(part 1 of 2)
# Autodesk Inventor assembly: Raspberry_Pi4 v19
Saved by Autodesk Inventor 2021.3 (Build 253353000, 353)
## iProperties
Created: 2023-06-15
Part Number: Raspberry_Pi4 v19
Document SubType Name: Assembly
Designer: AdminForWorker
Title: Raspberry_Pi4 v19 v1
Author: AdminForWorker
## Documents named in this file (370)
- z:\worker\convert-fusion-r02-cosv3\tmp\job-1\86\output\files\932a8257-b544-4e70-8857-ce00fc62fffb\fd29544b-6eeb-4b26-ae93-db3abaadae4f.iam
- z:\worker\convert-fusion-r02-cosv3\tmp\job-1\86\output\files\932a8257-b544-4e70-8857-ce00fc62fffb\Raspberry Pi 3157.ipt
- z:\worker\convert-fusion-r02-cosv3\tmp\job-1\86\output\files\932a8257-b544-4e70-8857-ce00fc62fffb\Raspberry Pi 3236.ipt
- z:\worker\convert-fusion-r02-cosv3\tmp\job-1\86\output\files\932a8257-b544-4e70-8857-ce00fc62fffb\Raspberry Pi 3237.ipt
- z:\worker\convert-fusion-r02-cosv3\tmp\job-1\86\output\files\932a8257-b544-4e70-8857-ce00fc62fffb\Raspberry Pi 3238.ipt
- z:\worker\convert-fusion-r02-cosv3\tmp\job-1\86\output\files\932a8257-b544-4e70-8857-ce00fc62fffb\Raspberry Pi 3239.ipt
- z:\worker\convert-fusion-r02-cosv3\tmp\job-1\86\output\files\932a8257-b544-4e70-8857-ce00fc62fffb\Raspberry Pi 3240.ipt
- z:\worker\convert-fusion-r02-cosv3\tmp\job-1\86\output\files\932a8257-b544-4e70-8857-ce00fc62fffb\Raspberry Pi 3241.ipt
- z:\worker\convert-fusion-r02-cosv3\tmp\job-1\86\output\files\932a8257-b544-4e70-8857-ce00fc62fffb\Raspberry Pi 3242.ipt
- z:\worker\convert-fusion-r02-cosv3\tmp\job-1\86\output\files\932a8257-b544-4e70-8857-ce00fc62fffb\Raspberry Pi 3243.ipt
- z:\worker\convert-fusion-r02-cosv3\tmp\job-1\86\output\files\932a8257-b544-4e70-8857-ce00fc62fffb\Raspberry Pi 3244.ipt
- z:\worker\convert-fusion-r02-cosv3\tmp\job-1\86\output\files\932a8257-b544-4e70-8857-ce00fc62fffb\Raspberry Pi 3245.ipt
- z:\worker\convert-fusion-r02-cosv3\tmp\job-1\86\output\files\932a8257-b544-4e70-8857-ce00fc62fffb\Raspberry Pi 3246.ipt
- z:\worker\convert-fusion-r02-cosv3\tmp\job-1\86\output\files\932a8257-b544-4e70-8857-ce00fc62fffb\Raspberry Pi 3247.ipt
- z:\worker\convert-fusion-r02-cosv3\tmp\job-1\86\output\files\932a8257-b544-4e70-8857-ce00fc62fffb\Raspberry Pi 3248.ipt
- z:\worker\convert-fusion-r02-cosv3\tmp\job-1\86\output\files\932a8257-b544-4e70-8857-ce00fc62fffb\Raspberry Pi 3249.ipt
- z:\worker\convert-fusion-r02-cosv3\tmp\job-1\86\output\files\932a8257-b544-4e70-8857-ce00fc62fffb\Raspberry Pi 3250.ipt
- z:\worker\convert-fusion-r02-cosv3\tmp\job-1\86\output\files\932a8257-b544-4e70-8857-ce00fc62fffb\Raspberry Pi 3251.ipt
- z:\worker\convert-fusion-r02-cosv3\tmp\job-1\86\output\files\932a8257-b544-4e70-8857-ce00fc62fffb\Raspberry Pi 3252.ipt
- z:\worker\convert-fusion-r02-cosv3\tmp\job-1\86\output\files\932a8257-b544-4e70-8857-ce00fc62fffb\Raspberry Pi 3253.ipt
- z:\worker\convert-fusion-r02-cosv3\tmp\job-1\86\output\files\932a8257-b544-4e70-8857-ce00fc62fffb\Raspberry Pi 3254.ipt
- z:\worker\convert-fusion-r02-cosv3\tmp\job-1\86\output\files\932a8257-b544-4e70-8857-ce00fc62fffb\Raspberry Pi 3255.ipt
- z:\worker\convert-fusion-r02-cosv3\tmp\job-1\86\output\files\932a8257-b544-4e70-8857-ce00fc62fffb\Raspberry Pi 3256.ipt
- z:\worker\convert-fusion-r02-cosv3\tmp\job-1\86\output\files\932a8257-b544-4e70-8857-ce00fc62fffb\Raspberry Pi 3257.ipt
- z:\worker\convert-fusion-r02-cosv3\tmp\job-1\86\output\files\932a8257-b544-4e70-8857-ce00fc62fffb\Raspberry Pi 3258.ipt
- z:\worker\convert-fusion-r02-cosv3\tmp\job-1\86\output\files\932a8257-b544-4e70-8857-ce00fc62fffb\Raspberry Pi 3259.ipt
- z:\worker\convert-fusion-r02-cosv3\tmp\job-1\86\output\files\932a8257-b544-4e70-8857-ce00fc62fffb\Raspberry Pi 3260.ipt
- z:\worker\convert-fusion-r02-cosv3\tmp\job-1\86\output\files\932a8257-b544-4e70-8857-ce00fc62fffb\Raspberry Pi 3261.ipt
- z:\worker\convert-fusion-r02-cosv3\tmp\job-1\86\output\files\932a8257-b544-4e70-8857-ce00fc62fffb\Raspberry Pi 3262.ipt
- z:\worker\convert-fusion-r02-cosv3\tmp\job-1\86\output\files\932a8257-b544-4e70-8857-ce00fc62fffb\Raspberry Pi 3263.ipt
- z:\worker\convert-fusion-r02-cosv3\tmp\job-1\86\output\files\932a8257-b544-4e70-8857-ce00fc62fffb\Raspberry Pi 3264.ipt
- z:\worker\convert-fusion-r02-cosv3\tmp\job-1\86\output\files\932a8257-b544-4e70-8857-ce00fc62fffb\Raspberry Pi 3265.ipt
- z:\worker\convert-fusion-r02-cosv3\tmp\job-1\86\output\files\932a8257-b544-4e70-8857-ce00fc62fffb\Raspberry Pi 3266.ipt
- z:\worker\convert-fusion-r02-cosv3\tmp\job-1\86\output\files\932a8257-b544-4e70-8857-ce00fc62fffb\Raspberry Pi 3267.ipt
- z:\worker\convert-fusion-r02-cosv3\tmp\job-1\86\output\files\932a8257-b544-4e70-8857-ce00fc62fffb\Raspberry Pi 3268.ipt
- z:\worker\convert-fusion-r02-cosv3\tmp\job-1\86\output\files\932a8257-b544-4e70-8857-ce00fc62fffb\Raspberry Pi 3269.ipt
- z:\worker\convert-fusion-r02-cosv3\tmp\job-1\86\output\files\932a8257-b544-4e70-8857-ce00fc62fffb\Raspberry Pi 3270.ipt
- z:\worker\convert-fusion-r02-cosv3\tmp\job-1\86\output\files\932a8257-b544-4e70-8857-ce00fc62fffb\Raspberry Pi 3271.ipt
- z:\worker\convert-fusion-r02-cosv3\tmp\job-1\86\output\files\932a8257-b544-4e70-8857-ce00fc62fffb\Raspberry Pi 3272.ipt
- z:\worker\convert-fusion-r02-cosv3\tmp\job-1\86\output\files\932a8257-b544-4e70-8857-ce00fc62fffb\Raspberry Pi 3273.ipt
- z:\worker\convert-fusion-r02-cosv3\tmp\job-1\86\output\files\932a8257-b544-4e70-8857-ce00fc62fffb\Raspberry Pi 3274.ipt
- z:\worker\convert-fusion-r02-cosv3\tmp\job-1\86\output\files\932a8257-b544-4e70-8857-ce00fc62fffb\Raspberry Pi 3275.ipt
- z:\worker\convert-fusion-r02-cosv3\tmp\job-1\86\output\files\932a8257-b544-4e70-8857-ce00fc62fffb\RPi3_ModelB v1.iam
- z:\worker\convert-fusion-r02-cosv3\tmp\job-1\86\output\files\932a8257-b544-4e70-8857-ce00fc62fffb\Raspberry Pi 312.ipt
- z:\worker\convert-fusion-r02-cosv3\tmp\job-1\86\output\files\932a8257-b544-4e70-8857-ce00fc62fffb\Raspberry Pi 314.ipt
- z:\worker\convert-fusion-r02-cosv3\tmp\job-1\86\output\files\932a8257-b544-4e70-8857-ce00fc62fffb\Raspberry Pi 3172.ipt
- z:\worker\convert-fusion-r02-cosv3\tmp\job-1\86\output\files\932a8257-b544-4e70-8857-ce00fc62fffb\Raspberry Pi 3173.ipt
- z:\worker\convert-fusion-r02-cosv3\tmp\job-1\86\output\files\932a8257-b544-4e70-8857-ce00fc62fffb\Raspberry Pi 3174.ipt
- z:\worker\convert-fusion-r02-cosv3\tmp\job-1\86\output\files\932a8257-b544-4e70-8857-ce00fc62fffb\Raspberry Pi 3175.ipt
- z:\worker\convert-fusion-r02-cosv3\tmp\job-1\86\output\files\932a8257-b544-4e70-8857-ce00fc62fffb\Raspberry Pi 3176.ipt
- z:\worker\convert-fusion-r02-cosv3\tmp\job-1\86\output\files\932a8257-b544-4e70-8857-ce00fc62fffb\Raspberry Pi 3177.ipt
- z:\worker\convert-fusion-r02-cosv3\tmp\job-1\86\output\files\932a8257-b544-4e70-8857-ce00fc62fffb\Raspberry Pi 3178.ipt
- z:\worker\convert-fusion-r02-cosv3\tmp\job-1\86\output\files\932a8257-b544-4e70-8857-ce00fc62fffb\Raspberry Pi 3179.ipt
- z:\worker\convert-fusion-r02-cosv3\tmp\job-1\86\output\files\932a8257-b544-4e70-8857-ce00fc62fffb\Raspberry Pi 3180.ipt
- z:\worker\convert-fusion-r02-cosv3\tmp\job-1\86\output\files\932a8257-b544-4e70-8857-ce00fc62fffb\Raspberry Pi 3181.ipt
- z:\worker\convert-fusion-r02-cosv3\tmp\job-1\86\output\files\932a8257-b544-4e70-8857-ce00fc62fffb\Raspberry Pi 3182.ipt
- z:\worker\convert-fusion-r02-cosv3\tmp\job-1\86\output\files\932a8257-b544-4e70-8857-ce00fc62fffb\Raspberry Pi 3183.ipt
- z:\worker\convert-fusion-r02-cosv3\tmp\job-1\86\output\files\932a8257-b544-4e70-8857-ce00fc62fffb\Raspberry Pi 3184.ipt
- z:\worker\convert-fusion-r02-cosv3\tmp\job-1\86\output\files\932a8257-b544-4e70-8857-ce00fc62fffb\Raspberry Pi 3185.ipt
- z:\worker\convert-fusion-r02-cosv3\tmp\job-1\86\output\files\932a8257-b544-4e70-8857-ce00fc62fffb\Raspberry Pi 3186.ipt
- z:\worker\convert-fusion-r02-cosv3\tmp\job-1\86\output\files\932a8257-b544-4e70-8857-ce00fc62fffb\Raspberry Pi 3187.ipt
- z:\worker\convert-fusion-r02-cosv3\tmp\job-1\86\output\files\932a8257-b544-4e70-8857-ce00fc62fffb\Raspberry Pi 3188.ipt
- z:\worker\convert-fusion-r02-cosv3\tmp\job-1\86\output\files\932a8257-b544-4e70-8857-ce00fc62fffb\Raspberry Pi 3189.ipt
- z:\worker\convert-fusion-r02-cosv3\tmp\job-1\86\output\files\932a8257-b544-4e70-8857-ce00fc62fffb\Raspberry Pi 3190.ipt
- z:\worker\convert-fusion-r02-cosv3\tmp\job-1\86\output\files\932a8257-b544-4e70-8857-ce00fc62fffb\Raspberry Pi 3191.ipt
- z:\worker\convert-fusion-r02-cosv3\tmp\job-1\86\output\files\932a8257-b544-4e70-8857-ce00fc62fffb\Raspberry Pi 3192.ipt
- z:\worker\convert-fusion-r02-cosv3\tmp\job-1\86\output\files\932a8257-b544-4e70-8857-ce00fc62fffb\Raspberry Pi 3193.ipt
- z:\worker\convert-fusion-r02-cosv3\tmp\job-1\86\output\files\932a8257-b544-4e70-8857-ce00fc62fffb\Raspberry Pi 3194.ipt
- z:\worker\convert-fusion-r02-cosv3\tmp\job-1\86\output\files\932a8257-b544-4e70-8857-ce00fc62fffb\Raspberry Pi 3195.ipt
- z:\worker\convert-fusion-r02-cosv3\tmp\job-1\86\output\files\932a8257-b544-4e70-8857-ce00fc62fffb\Raspberry Pi 3196.ipt
- z:\worker\convert-fusion-r02-cosv3\tmp\job-1\86\output\files\932a8257-b544-4e70-8857-ce00fc62fffb\Raspberry Pi 3197.ipt
- z:\worker\convert-fusion-r02-cosv3\tmp\job-1\86\output\files\932a8257-b544-4e70-8857-ce00fc62fffb\Raspberry Pi 3198.ipt
- z:\worker\convert-fusion-r02-cosv3\tmp\job-1\86\output\files\932a8257-b544-4e70-8857-ce00fc62fffb\Raspberry Pi 3199.ipt
- z:\worker\convert-fusion-r02-cosv3\tmp\job-1\86\output\files\932a8257-b544-4e70-8857-ce00fc62fffb\Raspberry Pi 3200.ipt
- z:\worker\convert-fusion-r02-cosv3\tmp\job-1\86\output\files\932a8257-b544-4e70-8857-ce00fc62fffb\Raspberry Pi 3201.ipt
- z:\worker\convert-fusion-r02-cosv3\tmp\job-1\86\output\files\932a8257-b544-4e70-8857-ce00fc62fffb\Raspberry Pi 3202.ipt
- z:\worker\convert-fusion-r02-cosv3\tmp\job-1\86\output\files\932a8257-b544-4e70-8857-ce00fc62fffb\Raspberry Pi 3203.ipt
- z:\worker\convert-fusion-r02-cosv3\tmp\job-1\86\output\files\932a8257-b544-4e70-8857-ce00fc62fffb\Raspberry Pi 3204.ipt
- z:\worker\convert-fusion-r02-cosv3\tmp\job-1\86\output\files\932a8257-b544-4e70-8857-ce00fc62fffb\Raspberry Pi 3205.ipt
- z:\worker\convert-fusion-r02-cosv3\tmp\job-1\86\output\files\932a8257-b544-4e70-8857-ce00fc62fffb\Raspberry Pi 3206.ipt
- z:\worker\convert-fusion-r02-cosv3\tmp\job-1\86\output\files\932a8257-b544-4e70-8857-ce00fc62fffb\Raspberry Pi 3207.ipt
- z:\worker\convert-fusion-r02-cosv3\tmp\job-1\86\output\files\932a8257-b544-4e70-8857-ce00fc62fffb\Raspberry Pi 3208.ipt
- z:\worker\convert-fusion-r02-cosv3\tmp\job-1\86\output\files\932a8257-b544-4e70-8857-ce00fc62fffb\Raspberry Pi 3209.ipt
- z:\worker\convert-fusion-r02-cosv3\tmp\job-1\86\output\files\932a8257-b544-4e70-8857-ce00fc62fffb\Raspberry Pi 3210.ipt
- z:\worker\convert-fusion-r02-cosv3\tmp\job-1\86\output\files\932a8257-b544-4e70-8857-ce00fc62fffb\Raspberry Pi 3211.ipt
- z:\worker\convert-fusion-r02-cosv3\tmp\job-1\86\output\files\932a8257-b544-4e70-8857-ce00fc62fffb\Raspberry Pi 3212.ipt
- z:\worker\convert-fusion-r02-cosv3\tmp\job-1\86\output\files\932a8257-b544-4e70-8857-ce00fc62fffb\Raspberry Pi 3213.ipt
- z:\worker\convert-fusion-r02-cosv3\tmp\job-1\86\output\files\932a8257-b544-4e70-8857-ce00fc62fffb\Raspberry Pi 3214.ipt
- z:\worker\convert-fusion-r02-cosv3\tmp\job-1\86\output\files\932a8257-b544-4e70-8857-ce00fc62fffb\Raspberry Pi 3215.ipt
- z:\worker\convert-fusion-r02-cosv3\tmp\job-1\86\output\files\932a8257-b544-4e70-8857-ce00fc62fffb\Raspberry Pi 3216.ipt
- z:\worker\convert-fusion-r02-cosv3\tmp\job-1\86\output\files\932a8257-b544-4e70-8857-ce00fc62fffb\Raspberry Pi 3217.ipt
- z:\worker\convert-fusion-r02-cosv3\tmp\job-1\86\output\files\932a8257-b544-4e70-8857-ce00fc62fffb\Raspberry Pi 3218.ipt
- z:\worker\convert-fusion-r02-cosv3\tmp\job-1\86\output\files\932a8257-b544-4e70-8857-ce00fc62fffb\Raspberry Pi 3219.ipt
- z:\worker\convert-fusion-r02-cosv3\tmp\job-1\86\output\files\932a8257-b544-4e70-8857-ce00fc62fffb\Raspberry Pi 3220.ipt
- z:\worker\convert-fusion-r02-cosv3\tmp\job-1\86\output\files\932a8257-b544-4e70-8857-ce00fc62fffb\Raspberry Pi 3221.ipt
- z:\worker\convert-fusion-r02-cosv3\tmp\job-1\86\output\files\932a8257-b544-4e70-8857-ce00fc62fffb\Raspberry Pi 3222.ipt
- z:\worker\convert-fusion-r02-cosv3\tmp\job-1\86\output\files\932a8257-b544-4e70-8857-ce00fc62fffb\Raspberry Pi 3223.ipt
- z:\worker\convert-fusion-r02-cosv3\tmp\job-1\86\output\files\932a8257-b544-4e70-8857-ce00fc62fffb\Raspberry Pi 3224.ipt
- z:\worker\convert-fusion-r02-cosv3\tmp\job-1\86\output\files\932a8257-b544-4e70-8857-ce00fc62fffb\Raspberry Pi 3225.ipt
- z:\worker\convert-fusion-r02-cosv3\tmp\job-1\86\output\files\932a8257-b544-4e70-8857-ce00fc62fffb\Raspberry Pi 3226.ipt
- z:\worker\convert-fusion-r02-cosv3\tmp\job-1\86\output\files\932a8257-b544-4e70-8857-ce00fc62fffb\Raspberry Pi 3227.ipt
- z:\worker\convert-fusion-r02-cosv3\tmp\job-1\86\output\files\932a8257-b544-4e70-8857-ce00fc62fffb\Raspberry Pi 3228.ipt
- z:\worker\convert-fusion-r02-cosv3\tmp\job-1\86\output\files\932a8257-b544-4e70-8857-ce00fc62fffb\Raspberry Pi 3229.ipt
- z:\worker\convert-fusion-r02-cosv3\tmp\job-1\86\output\files\932a8257-b544-4e70-8857-ce00fc62fffb\Raspberry Pi 3230.ipt
- z:\worker\convert-fusion-r02-cosv3\tmp\job-1\86\output\files\932a8257-b544-4e70-8857-ce00fc62fffb\Raspberry Pi 3231.ipt
- z:\worker\convert-fusion-r02-cosv3\tmp\job-1\86\output\files\932a8257-b544-4e70-8857-ce00fc62fffb\Raspberry Pi 3232.ipt
- z:\worker\convert-fusion-r02-cosv3\tmp\job-1\86\output\files\932a8257-b544-4e70-8857-ce00fc62fffb\Raspberry Pi 3233.ipt
- z:\worker\convert-fusion-r02-cosv3\tmp\job-1\86\output\files\932a8257-b544-4e70-8857-ce00fc62fffb\Raspberry Pi 3234.ipt
- z:\worker\convert-fusion-r02-cosv3\tmp\job-1\86\output\files\932a8257-b544-4e70-8857-ce00fc62fffb\Raspberry Pi 3235.ipt
- z:\worker\convert-fusion-r02-cosv3\tmp\job-1\86\output\files\932a8257-b544-4e70-8857-ce00fc62fffb\Raspberry Pi 31.ipt
- z:\worker\convert-fusion-r02-cosv3\tmp\job-1\86\output\files\932a8257-b544-4e70-8857-ce00fc62fffb\Raspberry Pi 32.ipt
- z:\worker\convert-fusion-r02-cosv3\tmp\job-1\86\output\files\932a8257-b544-4e70-8857-ce00fc62fffb\Raspberry Pi 33.ipt
- z:\worker\convert-fusion-r02-cosv3\tmp\job-1\86\output\files\932a8257-b544-4e70-8857-ce00fc62fffb\Raspberry Pi 34.ipt
- z:\worker\convert-fusion-r02-cosv3\tmp\job-1\86\output\files\932a8257-b544-4e70-8857-ce00fc62fffb\Raspberry Pi 35.ipt
- z:\worker\convert-fusion-r02-cosv3\tmp\job-1\86\output\files\932a8257-b544-4e70-8857-ce00fc62fffb\Raspberry Pi 36.ipt
- z:\worker\convert-fusion-r02-cosv3\tmp\job-1\86\output\files\932a8257-b544-4e70-8857-ce00fc62fffb\Raspberry Pi 37.ipt
- z:\worker\convert-fusion-r02-cosv3\tmp\job-1\86\output\files\932a8257-b544-4e70-8857-ce00fc62fffb\Raspberry Pi 38.ipt
- z:\worker\convert-fusion-r02-cosv3\tmp\job-1\86\output\files\932a8257-b544-4e70-8857-ce00fc62fffb\Raspberry Pi 39.ipt
- z:\worker\convert-fusion-r02-cosv3\tmp\job-1\86\output\files\932a8257-b544-4e70-8857-ce00fc62fffb\Raspberry Pi 310.ipt
- z:\worker\convert-fusion-r02-cosv3\tmp\job-1\86\output\files\932a8257-b544-4e70-8857-ce00fc62fffb\Raspberry Pi 311.ipt
- z:\worker\convert-fusion-r02-cosv3\tmp\job-1\86\output\files\932a8257-b544-4e70-8857-ce00fc62fffb\Raspberry Pi 313.ipt
- z:\worker\convert-fusion-r02-cosv3\tmp\job-1\86\output\files\932a8257-b544-4e70-8857-ce00fc62fffb\Raspberry Pi 315.ipt
- z:\worker\convert-fusion-r02-cosv3\tmp\job-1\86\output\files\932a8257-b544-4e70-8857-ce00fc62fffb\Raspberry Pi 316.ipt
- z:\worker\convert-fusion-r02-cosv3\tmp\job-1\86\output\files\932a8257-b544-4e70-8857-ce00fc62fffb\Raspberry Pi 317.ipt
- z:\worker\convert-fusion-r02-cosv3\tmp\job-1\86\output\files\932a8257-b544-4e70-8857-ce00fc62fffb\Raspberry Pi 318.ipt
- z:\worker\convert-fusion-r02-cosv3\tmp\job-1\86\output\files\932a8257-b544-4e70-8857-ce00fc62fffb\Raspberry Pi 319.ipt
- z:\worker\convert-fusion-r02-cosv3\tmp\job-1\86\output\files\932a8257-b544-4e70-8857-ce00fc62fffb\Raspberry Pi 320.ipt
- z:\worker\convert-fusion-r02-cosv3\tmp\job-1\86\output\files\932a8257-b544-4e70-8857-ce00fc62fffb\Raspberry Pi 322.ipt
- z:\worker\convert-fusion-r02-cosv3\tmp\job-1\86\output\files\932a8257-b544-4e70-8857-ce00fc62fffb\Raspberry Pi 323.ipt
- z:\worker\convert-fusion-r02-cosv3\tmp\job-1\86\output\files\932a8257-b544-4e70-8857-ce00fc62fffb\Raspberry Pi 324.ipt
- z:\worker\convert-fusion-r02-cosv3\tmp\job-1\86\output\files\932a8257-b544-4e70-8857-ce00fc62fffb\Raspberry Pi 325.ipt
- z:\worker\convert-fusion-r02-cosv3\tmp\job-1\86\output\files\932a8257-b544-4e70-8857-ce00fc62fffb\Raspberry Pi 326.ipt
- z:\worker\convert-fusion-r02-cosv3\tmp\job-1\86\output\files\932a8257-b544-4e70-8857-ce00fc62fffb\Raspberry Pi 327.ipt
- z:\worker\convert-fusion-r02-cosv3\tmp\job-1\86\output\files\932a8257-b544-4e70-8857-ce00fc62fffb\Raspberry Pi 328.ipt
- z:\worker\convert-fusion-r02-cosv3\tmp\job-1\86\output\files\932a8257-b544-4e70-8857-ce00fc62fffb\Raspberry Pi 329.ipt
- z:\worker\convert-fusion-r02-cosv3\tmp\job-1\86\output\files\932a8257-b544-4e70-8857-ce00fc62fffb\Raspberry Pi 330.ipt
- z:\worker\convert-fusion-r02-cosv3\tmp\job-1\86\output\files\932a8257-b544-4e70-8857-ce00fc62fffb\Raspberry Pi 331.ipt
- z:\worker\convert-fusion-r02-cosv3\tmp\job-1\86\output\files\932a8257-b544-4e70-8857-ce00fc62fffb\Raspberry Pi 332.ipt
- z:\worker\convert-fusion-r02-cosv3\tmp\job-1\86\output\files\932a8257-b544-4e70-8857-ce00fc62fffb\Raspberry Pi 333.ipt
- z:\worker\convert-fusion-r02-cosv3\tmp\job-1\86\output\files\932a8257-b544-4e70-8857-ce00fc62fffb\Raspberry Pi 334.ipt
- z:\worker\convert-fusion-r02-cosv3\tmp\job-1\86\output\files\932a8257-b544-4e70-8857-ce00fc62fffb\Raspberry Pi 335.ipt
- z:\worker\convert-fusion-r02-cosv3\tmp\job-1\86\output\files\932a8257-b544-4e70-8857-ce00fc62fffb\Raspberry Pi 336.ipt
- z:\worker\convert-fusion-r02-cosv3\tmp\job-1\86\output\files\932a8257-b544-4e70-8857-ce00fc62fffb\Raspberry Pi 337.ipt
- z:\worker\convert-fusion-r02-cosv3\tmp\job-1\86\output\files\932a8257-b544-4e70-8857-ce00fc62fffb\Raspberry Pi 338.ipt
- z:\worker\convert-fusion-r02-cosv3\tmp\job-1\86\output\files\932a8257-b544-4e70-8857-ce00fc62fffb\Raspberry Pi 339.ipt
- z:\worker\convert-fusion-r02-cosv3\tmp\job-1\86\output\files\932a8257-b544-4e70-8857-ce00fc62fffb\Raspberry Pi 340.ipt
- z:\worker\convert-fusion-r02-cosv3\tmp\job-1\86\output\files\932a8257-b544-4e70-8857-ce00fc62fffb\Raspberry Pi 341.ipt
- z:\worker\convert-fusion-r02-cosv3\tmp\job-1\86\output\files\932a8257-b544-4e70-8857-ce00fc62fffb\Raspberry Pi 342.ipt
- z:\worker\convert-fusion-r02-cosv3\tmp\job-1\86\output\files\932a8257-b544-4e70-8857-ce00fc62fffb\Raspberry Pi 343.ipt
- z:\worker\convert-fusion-r02-cosv3\tmp\job-1\86\output\files\932a8257-b544-4e70-8857-ce00fc62fffb\Raspberry Pi 344.ipt
- z:\worker\convert-fusion-r02-cosv3\tmp\job-1\86\output\files\932a8257-b544-4e70-8857-ce00fc62fffb\Raspberry Pi 345.ipt
- z:\worker\convert-fusion-r02-cosv3\tmp\job-1\86\output\files\932a8257-b544-4e70-8857-ce00fc62fffb\Raspberry Pi 346.ipt
- z:\worker\convert-fusion-r02-cosv3\tmp\job-1\86\output\files\932a8257-b544-4e70-8857-ce00fc62fffb\Raspberry Pi 347.ipt
- z:\worker\convert-fusion-r02-cosv3\tmp\job-1\86\output\files\932a8257-b544-4e70-8857-ce00fc62fffb\Raspberry Pi 348.ipt
- z:\worker\convert-fusion-r02-cosv3\tmp\job-1\86\output\files\932a8257-b544-4e70-8857-ce00fc62fffb\Raspberry Pi 349.ipt
- z:\worker\convert-fusion-r02-cosv3\tmp\job-1\86\output\files\932a8257-b544-4e70-8857-ce00fc62fffb\Raspberry Pi 350.ipt
- z:\worker\convert-fusion-r02-cosv3\tmp\job-1\86\output\files\932a8257-b544-4e70-8857-ce00fc62fffb\Raspberry Pi 351.ipt
- z:\worker\convert-fusion-r02-cosv3\tmp\job-1\86\output\files\932a8257-b544-4e70-8857-ce00fc62fffb\Raspberry Pi 352.ipt
- z:\worker\convert-fusion-r02-cosv3\tmp\job-1\86\output\files\932a8257-b544-4e70-8857-ce00fc62fffb\Raspberry Pi 353.ipt
- z:\worker\convert-fusion-r02-cosv3\tmp\job-1\86\output\files\932a8257-b544-4e70-8857-ce00fc62fffb\Raspberry Pi 354.ipt
- z:\worker\convert-fusion-r02-cosv3\tmp\job-1\86\output\files\932a8257-b544-4e70-8857-ce00fc62fffb\Raspberry Pi 355.ipt
- z:\worker\convert-fusion-r02-cosv3\tmp\job-1\86\output\files\932a8257-b544-4e70-8857-ce00fc62fffb\Raspberry Pi 356.ipt
- z:\worker\convert-fusion-r02-cosv3\tmp\job-1\86\output\files\932a8257-b544-4e70-8857-ce00fc62fffb\Raspberry Pi 357.ipt
- z:\worker\convert-fusion-r02-cosv3\tmp\job-1\86\output\files\932a8257-b544-4e70-8857-ce00fc62fffb\Raspberry Pi 358.ipt
- z:\worker\convert-fusion-r02-cosv3\tmp\job-1\86\output\files\932a8257-b544-4e70-8857-ce00fc62fffb\Raspberry Pi 359.ipt
- z:\worker\convert-fusion-r02-cosv3\tmp\job-1\86\output\files\932a8257-b544-4e70-8857-ce00fc62fffb\Raspberry Pi 360.ipt
- z:\worker\convert-fusion-r02-cosv3\tmp\job-1\86\output\files\932a8257-b544-4e70-8857-ce00fc62fffb\Raspberry Pi 361.ipt
- z:\worker\convert-fusion-r02-cosv3\tmp\job-1\86\output\files\932a8257-b544-4e70-8857-ce00fc62fffb\Raspberry Pi 362.ipt
- z:\worker\convert-fusion-r02-cosv3\tmp\job-1\86\output\files\932a8257-b544-4e70-8857-ce00fc62fffb\Raspberry Pi 363.ipt
- z:\worker\convert-fusion-r02-cosv3\tmp\job-1\86\output\files\932a8257-b544-4e70-8857-ce00fc62fffb\Raspberry Pi 364.ipt
- z:\worker\convert-fusion-r02-cosv3\tmp\job-1\86\output\files\932a8257-b544-4e70-8857-ce00fc62fffb\Raspberry Pi 365.ipt
- z:\worker\convert-fusion-r02-cosv3\tmp\job-1\86\output\files\932a8257-b544-4e70-8857-ce00fc62fffb\Raspberry Pi 366.ipt
- z:\worker\convert-fusion-r02-cosv3\tmp\job-1\86\output\files\932a8257-b544-4e70-8857-ce00fc62fffb\Raspberry Pi 367.ipt
- z:\worker\convert-fusion-r02-cosv3\tmp\job-1\86\output\files\932a8257-b544-4e70-8857-ce00fc62fffb\Raspberry Pi 368.ipt
- z:\worker\convert-fusion-r02-cosv3\tmp\job-1\86\output\files\932a8257-b544-4e70-8857-ce00fc62fffb\Raspberry Pi 369.ipt
- z:\worker\convert-fusion-r02-cosv3\tmp\job-1\86\output\files\932a8257-b544-4e70-8857-ce00fc62fffb\Raspberry Pi 370.ipt
- z:\worker\convert-fusion-r02-cosv3\tmp\job-1\86\output\files\932a8257-b544-4e70-8857-ce00fc62fffb\Raspberry Pi 371.ipt
- z:\worker\convert-fusion-r02-cosv3\tmp\job-1\86\output\files\932a8257-b544-4e70-8857-ce00fc62fffb\Raspberry Pi 372.ipt
- z:\worker\convert-fusion-r02-cosv3\tmp\job-1\86\output\files\932a8257-b544-4e70-8857-ce00fc62fffb\Raspberry Pi 373.ipt
- z:\worker\convert-fusion-r02-cosv3\tmp\job-1\86\output\files\932a8257-b544-4e70-8857-ce00fc62fffb\Raspberry Pi 374.ipt
- z:\worker\convert-fusion-r02-cosv3\tmp\job-1\86\output\files\932a8257-b544-4e70-8857-ce00fc62fffb\Raspberry Pi 375.ipt
- z:\worker\convert-fusion-r02-cosv3\tmp\job-1\86\output\files\932a8257-b544-4e70-8857-ce00fc62fffb\Raspberry Pi 376.ipt
- z:\worker\convert-fusion-r02-cosv3\tmp\job-1\86\output\files\932a8257-b544-4e70-8857-ce00fc62fffb\Raspberry Pi 377.ipt
- z:\worker\convert-fusion-r02-cosv3\tmp\job-1\86\output\files\932a8257-b544-4e70-8857-ce00fc62fffb\Raspberry Pi 378.ipt
- z:\worker\convert-fusion-r02-cosv3\tmp\job-1\86\output\files\932a8257-b544-4e70-8857-ce00fc62fffb\Raspberry Pi 379.ipt
- z:\worker\convert-fusion-r02-cosv3\tmp\job-1\86\output\files\932a8257-b544-4e70-8857-ce00fc62fffb\Raspberry Pi 380.ipt
- z:\worker\convert-fusion-r02-cosv3\tmp\job-1\86\output\files\932a8257-b544-4e70-8857-ce00fc62fffb\Raspberry Pi 381.ipt
- z:\worker\convert-fusion-r02-cosv3\tmp\job-1\86\output\files\932a8257-b544-4e70-8857-ce00fc62fffb\Raspberry Pi 382.ipt
- z:\worker\convert-fusion-r02-cosv3\tmp\job-1\86\output\files\932a8257-b544-4e70-8857-ce00fc62fffb\Raspberry Pi 383.ipt
- z:\worker\convert-fusion-r02-cosv3\tmp\job-1\86\output\files\932a8257-b544-4e70-8857-ce00fc62fffb\Raspberry Pi 385.ipt
- z:\worker\convert-fusion-r02-cosv3\tmp\job-1\86\output\files\932a8257-b544-4e70-8857-ce00fc62fffb\Raspberry Pi 386.ipt
- z:\worker\convert-fusion-r02-cosv3\tmp\job-1\86\output\files\932a8257-b544-4e70-8857-ce00fc62fffb\Raspberry Pi 387.ipt
- z:\worker\convert-fusion-r02-cosv3\tmp\job-1\86\output\files\932a8257-b544-4e70-8857-ce00fc62fffb\Raspberry Pi 388.ipt
- z:\worker\convert-fusion-r02-cosv3\tmp\job-1\86\output\files\932a8257-b544-4e70-8857-ce00fc62fffb\Raspberry Pi 390.ipt
- z:\worker\convert-fusion-r02-cosv3\tmp\job-1\86\output\files\932a8257-b544-4e70-8857-ce00fc62fffb\Raspberry Pi 391.ipt
- z:\worker\convert-fusion-r02-cosv3\tmp\job-1\86\output\files\932a8257-b544-4e70-8857-ce00fc62fffb\Raspberry Pi 393.ipt
- z:\worker\convert-fusion-r02-cosv3\tmp\job-1\86\output\files\932a8257-b544-4e70-8857-ce00fc62fffb\Raspberry Pi 394.ipt
- z:\worker\convert-fusion-r02-cosv3\tmp\job-1\86\output\files\932a8257-b544-4e70-8857-ce00fc62fffb\Raspberry Pi 395.ipt
- z:\worker\convert-fusion-r02-cosv3\tmp\job-1\86\output\files\932a8257-b544-4e70-8857-ce00fc62fffb\Raspberry Pi 396.ipt
- z:\worker\convert-fusion-r02-cosv3\tmp\job-1\86\output\files\932a8257-b544-4e70-8857-ce00fc62fffb\Raspberry Pi 397.ipt
- z:\worker\convert-fusion-r02-cosv3\tmp\job-1\86\output\files\932a8257-b544-4e70-8857-ce00fc62fffb\Raspberry Pi 398.ipt
- z:\worker\convert-fusion-r02-cosv3\tmp\job-1\86\output\files\932a8257-b544-4e70-8857-ce00fc62fffb\Raspberry Pi 399.ipt
- z:\worker\convert-fusion-r02-cosv3\tmp\job-1\86\output\files\932a8257-b544-4e70-8857-ce00fc62fffb\Raspberry Pi 3100.ipt
- z:\worker\convert-fusion-r02-cosv3\tmp\job-1\86\output\files\932a8257-b544-4e70-8857-ce00fc62fffb\Raspberry Pi 3101.ipt
- z:\worker\convert-fusion-r02-cosv3\tmp\job-1\86\output\files\932a8257-b544-4e70-8857-ce00fc62fffb\Raspberry Pi 3102.ipt
- z:\worker\convert-fusion-r02-cosv3\tmp\job-1\86\output\files\932a8257-b544-4e70-8857-ce00fc62fffb\Raspberry Pi 3103.ipt
- z:\worker\convert-fusion-r02-cosv3\tmp\job-1\86\output\files\932a8257-b544-4e70-8857-ce00fc62fffb\Raspberry Pi 3104.ipt
- z:\worker\convert-fusion-r02-cosv3\tmp\job-1\86\output\files\932a8257-b544-4e70-8857-ce00fc62fffb\Raspberry Pi 3105.ipt
- z:\worker\convert-fusion-r02-cosv3\tmp\job-1\86\output\files\932a8257-b544-4e70-8857-ce00fc62fffb\Raspberry Pi 3106.ipt
- z:\worker\convert-fusion-r02-cosv3\tmp\job-1\86\output\files\932a8257-b544-4e70-8857-ce00fc62fffb\Raspberry Pi 3107.ipt
- z:\worker\convert-fusion-r02-cosv3\tmp\job-1\86\output\files\932a8257-b544-4e70-8857-ce00fc62fffb\Raspberry Pi 3108.ipt
- z:\worker\convert-fusion-r02-cosv3\tmp\job-1\86\output\files\932a8257-b544-4e70-8857-ce00fc62fffb\Raspberry Pi 3109.ipt
- z:\worker\convert-fusion-r02-cosv3\tmp\job-1\86\output\files\932a8257-b544-4e70-8857-ce00fc62fffb\Raspberry Pi 3110.ipt
- z:\worker\convert-fusion-r02-cosv3\tmp\job-1\86\output\files\932a8257-b544-4e70-8857-ce00fc62fffb\Raspberry Pi 3111.ipt
- z:\worker\convert-fusion-r02-cosv3\tmp\job-1\86\output\files\932a8257-b544-4e70-8857-ce00fc62fffb\Raspberry Pi 3112.ipt
- z:\worker\convert-fusion-r02-cosv3\tmp\job-1\86\output\files\932a8257-b544-4e70-8857-ce00fc62fffb\Raspberry Pi 3113.ipt
- z:\worker\convert-fusion-r02-cosv3\tmp\job-1\86\output\files\932a8257-b544-4e70-8857-ce00fc62fffb\Raspberry Pi 3114.ipt
- z:\worker\convert-fusion-r02-cosv3\tmp\job-1\86\output\files\932a8257-b544-4e70-8857-ce00fc62fffb\Raspberry Pi 3115.ipt
- z:\worker\convert-fusion-r02-cosv3\tmp\job-1\86\output\files\932a8257-b544-4e70-8857-ce00fc62fffb\Raspberry Pi 3116.ipt
- z:\worker\convert-fusion-r02-cosv3\tmp\job-1\86\output\files\932a8257-b544-4e70-8857-ce00fc62fffb\Raspberry Pi 3117.ipt
- z:\worker\convert-fusion-r02-cosv3\tmp\job-1\86\output\files\932a8257-b544-4e70-8857-ce00fc62fffb\Raspberry Pi 3118.ipt
- z:\worker\convert-fusion-r02-cosv3\tmp\job-1\86\output\files\932a8257-b544-4e70-8857-ce00fc62fffb\Raspberry Pi 3119.ipt
- z:\worker\convert-fusion-r02-cosv3\tmp\job-1\86\output\files\932a8257-b544-4e70-8857-ce00fc62fffb\Raspberry Pi 3120.ipt
- z:\worker\convert-fusion-r02-cosv3\tmp\job-1\86\output\files\932a8257-b544-4e70-8857-ce00fc62fffb\Raspberry Pi 3121.ipt
- z:\worker\convert-fusion-r02-cosv3\tmp\job-1\86\output\files\932a8257-b544-4e70-8857-ce00fc62fffb\Raspberry Pi 3122.ipt
- z:\worker\convert-fusion-r02-cosv3\tmp\job-1\86\output\files\932a8257-b544-4e70-8857-ce00fc62fffb\Raspberry Pi 3123.ipt
- z:\worker\convert-fusion-r02-cosv3\tmp\job-1\86\output\files\932a8257-b544-4e70-8857-ce00fc62fffb\Raspberry Pi 3124.ipt
- z:\worker\convert-fusion-r02-cosv3\tmp\job-1\86\output\files\932a8257-b544-4e70-8857-ce00fc62fffb\Raspberry Pi 3125.ipt
- z:\worker\convert-fusion-r02-cosv3\tmp\job-1\86\output\files\932a8257-b544-4e70-8857-ce00fc62fffb\Raspberry Pi 3126.ipt
- z:\worker\convert-fusion-r02-cosv3\tmp\job-1\86\output\files\932a8257-b544-4e70-8857-ce00fc62fffb\Raspberry Pi 3127.ipt
- z:\worker\convert-fusion-r02-cosv3\tmp\job-1\86\output\files\932a8257-b544-4e70-8857-ce00fc62fffb\Raspberry Pi 3128.ipt
- z:\worker\convert-fusion-r02-cosv3\tmp\job-1\86\output\files\932a8257-b544-4e70-8857-ce00fc62fffb\Raspberry Pi 3129.ipt
- z:\worker\convert-fusion-r02-cosv3\tmp\job-1\86\output\files\932a8257-b544-4e70-8857-ce00fc62fffb\Raspberry Pi 3130.ipt
- z:\worker\convert-fusion-r02-cosv3\tmp\job-1\86\output\files\932a8257-b544-4e70-8857-ce00fc62fffb\Raspberry Pi 3131.ipt
- z:\worker\convert-fusion-r02-cosv3\tmp\job-1\86\output\files\932a8257-b544-4e70-8857-ce00fc62fffb\Raspberry Pi 3132.ipt
- z:\worker\convert-fusion-r02-cosv3\tmp\job-1\86\output\files\932a8257-b544-4e70-8857-ce00fc62fffb\Raspberry Pi 3133.ipt
- z:\worker\convert-fusion-r02-cosv3\tmp\job-1\86\output\files\932a8257-b544-4e70-8857-ce00fc62fffb\Raspberry Pi 3134.ipt
- z:\worker\convert-fusion-r02-cosv3\tmp\job-1\86\output\files\932a8257-b544-4e70-8857-ce00fc62fffb\Raspberry Pi 3135.ipt
- z:\worker\convert-fusion-r02-cosv3\tmp\job-1\86\output\files\932a8257-b544-4e70-8857-ce00fc62fffb\Raspberry Pi 3137.ipt
- z:\worker\convert-fusion-r02-cosv3\tmp\job-1\86\output\files\932a8257-b544-4e70-8857-ce00fc62fffb\Raspberry Pi 3138.ipt
- z:\worker\convert-fusion-r02-cosv3\tmp\job-1\86\output\files\932a8257-b544-4e70-8857-ce00fc62fffb\Raspberry Pi 3139.ipt
- z:\worker\convert-fusion-r02-cosv3\tmp\job-1\86\output\files\932a8257-b544-4e70-8857-ce00fc62fffb\Raspberry Pi 3140.ipt
- z:\worker\convert-fusion-r02-cosv3\tmp\job-1\86\output\files\932a8257-b544-4e70-8857-ce00fc62fffb\Raspberry Pi 3141.ipt
- z:\worker\convert-fusion-r02-cosv3\tmp\job-1\86\output\files\932a8257-b544-4e70-8857-ce00fc62fffb\Raspberry Pi 3142.ipt
- z:\worker\convert-fusion-r02-cosv3\tmp\job-1\86\output\files\932a8257-b544-4e70-8857-ce00fc62fffb\Raspberry Pi 3143.ipt
- z:\worker\convert-fusion-r02-cosv3\tmp\job-1\86\output\files\932a8257-b544-4e70-8857-ce00fc62fffb\Raspberry Pi 3144.ipt
- z:\worker\convert-fusion-r02-cosv3\tmp\job-1\86\output\files\932a8257-b544-4e70-8857-ce00fc62fffb\Raspberry Pi 3146.ipt
- z:\worker\convert-fusion-r02-cosv3\tmp\job-1\86\output\files\932a8257-b544-4e70-8857-ce00fc62fffb\Raspberry Pi 3147.ipt
- z:\worker\convert-fusion-r02-cosv3\tmp\job-1\86\output\files\932a8257-b544-4e70-8857-ce00fc62fffb\Raspberry Pi 3149.ipt
- z:\worker\convert-fusion-r02-cosv3\tmp\job-1\86\output\files\932a8257-b544-4e70-8857-ce00fc62fffb\Raspberry Pi 3150.ipt
- z:\worker\convert-fusion-r02-cosv3\tmp\job-1\86\output\files\932a8257-b544-4e70-8857-ce00fc62fffb\Raspberry Pi 3151.ipt
- z:\worker\convert-fusion-r02-cosv3\tmp\job-1\86\output\files\932a8257-b544-4e70-8857-ce00fc62fffb\Raspberry Pi 3152.ipt
- z:\worker\convert-fusion-r02-cosv3\tmp\job-1\86\output\files\932a8257-b544-4e70-8857-ce00fc62fffb\Raspberry Pi 3153.ipt
- z:\worker\convert-fusion-r02-cosv3\tmp\job-1\86\output\files\932a8257-b544-4e70-8857-ce00fc62fffb\Raspberry Pi 3154.ipt
- z:\worker\convert-fusion-r02-cosv3\tmp\job-1\86\output\files\932a8257-b544-4e70-8857-ce00fc62fffb\Raspberry Pi 3155.ipt
- z:\worker\convert-fusion-r02-cosv3\tmp\job-1\86\output\files\932a8257-b544-4e70-8857-ce00fc62fffb\Raspberry Pi 3156.ipt
- z:\worker\convert-fusion-r02-cosv3\tmp\job-1\86\output\files\932a8257-b544-4e70-8857-ce00fc62fffb\Raspberry Pi 3158.ipt
- z:\worker\convert-fusion-r02-cosv3\tmp\job-1\86\output\files\932a8257-b544-4e70-8857-ce00fc62fffb\Raspberry Pi 3159.ipt
- z:\worker\convert-fusion-r02-cosv3\tmp\job-1\86\output\files\932a8257-b544-4e70-8857-ce00fc62fffb\Raspberry Pi 3160.ipt
- z:\worker\convert-fusion-r02-cosv3\tmp\job-1\86\output\files\932a8257-b544-4e70-8857-ce00fc62fffb\Raspberry Pi 3161.ipt
- z:\worker\convert-fusion-r02-cosv3\tmp\job-1\86\output\files\932a8257-b544-4e70-8857-ce00fc62fffb\Raspberry Pi 3162.ipt
- z:\worker\convert-fusion-r02-cosv3\tmp\job-1\86\output\files\932a8257-b544-4e70-8857-ce00fc62fffb\Raspberry Pi 3163.ipt
- z:\worker\convert-fusion-r02-cosv3\tmp\job-1\86\output\files\932a8257-b544-4e70-8857-ce00fc62fffb\Raspberry Pi 3164.ipt
- z:\worker\convert-fusion-r02-cosv3\tmp\job-1\86\output\files\932a8257-b544-4e70-8857-ce00fc62fffb\Raspberry Pi 3165.ipt
- z:\worker\convert-fusion-r02-cosv3\tmp\job-1\86\output\files\932a8257-b544-4e70-8857-ce00fc62fffb\Raspberry Pi 3166.ipt
- z:\worker\convert-fusion-r02-cosv3\tmp\job-1\86\output\files\932a8257-b544-4e70-8857-ce00fc62fffb\Raspberry Pi 3167.ipt
- z:\worker\convert-fusion-r02-cosv3\tmp\job-1\86\output\files\932a8257-b544-4e70-8857-ce00fc62fffb\Raspberry Pi 3168.ipt
- z:\worker\convert-fusion-r02-cosv3\tmp\job-1\86\output\files\932a8257-b544-4e70-8857-ce00fc62fffb\Raspberry Pi 3169.ipt
- z:\worker\convert-fusion-r02-cosv3\tmp\job-1\86\output\files\932a8257-b544-4e70-8857-ce00fc62fffb\Raspberry Pi 3170.ipt
- z:\worker\convert-fusion-r02-cosv3\tmp\job-1\86\output\files\932a8257-b544-4e70-8857-ce00fc62fffb\Raspberry Pi 3171.ipt
- z:\worker\convert-fusion-r02-cosv3\tmp\job-1\86\output\files\932a8257-b544-4e70-8857-ce00fc62fffb\Raspberry Pi 3276.ipt
- z:\worker\convert-fusion-r02-cosv3\tmp\job-1\86\output\files\932a8257-b544-4e70-8857-ce00fc62fffb\Raspberry Pi 3277.ipt
- z:\worker\convert-fusion-r02-cosv3\tmp\job-1\86\output\files\932a8257-b544-4e70-8857-ce00fc62fffb\Raspberry Pi 3278.ipt
- z:\worker\convert-fusion-r02-cosv3\tmp\job-1\86\output\files\932a8257-b544-4e70-8857-ce00fc62fffb\Raspberry Pi 3279.ipt
- z:\worker\convert-fusion-r02-cosv3\tmp\job-1\86\output\files\932a8257-b544-4e70-8857-ce00fc62fffb\Raspberry Pi 3280.ipt
- z:\worker\convert-fusion-r02-cosv3\tmp\job-1\86\output\files\932a8257-b544-4e70-8857-ce00fc62fffb\Raspberry Pi 3281.ipt
- z:\worker\convert-fusion-r02-cosv3\tmp\job-1\86\output\files\932a8257-b544-4e70-8857-ce00fc62fffb\Raspberry Pi 3282.ipt
- z:\worker\convert-fusion-r02-cosv3\tmp\job-1\86\output\files\932a8257-b544-4e70-8857-ce00fc62fffb\Raspberry Pi 3283.ipt
- z:\worker\convert-fusion-r02-cosv3\tmp\job-1\86\output\files\932a8257-b544-4e70-8857-ce00fc62fffb\Raspberry Pi 3284.ipt
- z:\worker\convert-fusion-r02-cosv3\tmp\job-1\86\output\files\932a8257-b544-4e70-8857-ce00fc62fffb\Raspberry Pi 3285.ipt
- z:\worker\convert-fusion-r02-cosv3\tmp\job-1\86\output\files\932a8257-b544-4e70-8857-ce00fc62fffb\Raspberry Pi 3286.ipt
- z:\worker\convert-fusion-r02-cosv3\tmp\job-1\86\output\files\932a8257-b544-4e70-8857-ce00fc62fffb\Raspberry Pi 3287.ipt
- z:\worker\convert-fusion-r02-cosv3\tmp\job-1\86\output\files\932a8257-b544-4e70-8857-ce00fc62fffb\Raspberry Pi 3288.ipt
- z:\worker\convert-fusion-r02-cosv3\tmp\job-1\86\output\files\932a8257-b544-4e70-8857-ce00fc62fffb\Raspberry Pi 3289.ipt
- z:\worker\convert-fusion-r02-cosv3\tmp\job-1\86\output\files\932a8257-b544-4e70-8857-ce00fc62fffb\Raspberry Pi 3290.ipt
- z:\worker\convert-fusion-r02-cosv3\tmp\job-1\86\output\files\932a8257-b544-4e70-8857-ce00fc62fffb\Raspberry Pi 3291.ipt
- z:\worker\convert-fusion-r02-cosv3\tmp\job-1\86\output\files\932a8257-b544-4e70-8857-ce00fc62fffb\Raspberry Pi 3292.ipt
- z:\worker\convert-fusion-r02-cosv3\tmp\job-1\86\output\files\932a8257-b544-4e70-8857-ce00fc62fffb\Raspberry Pi 3293.ipt
- z:\worker\convert-fusion-r02-cosv3\tmp\job-1\86\output\files\932a8257-b544-4e70-8857-ce00fc62fffb\Raspberry Pi 3294.ipt
- z:\worker\convert-fusion-r02-cosv3\tmp\job-1\86\output\files\932a8257-b544-4e70-8857-ce00fc62fffb\Raspberry Pi 3295.ipt
- z:\worker\convert-fusion-r02-cosv3\tmp\job-1\86\output\files\932a8257-b544-4e70-8857-ce00fc62fffb\Raspberry Pi 3296.ipt
- z:\worker\convert-fusion-r02-cosv3\tmp\job-1\86\output\files\932a8257-b544-4e70-8857-ce00fc62fffb\Raspberry Pi 3297.ipt
- z:\worker\convert-fusion-r02-cosv3\tmp\job-1\86\output\files\932a8257-b544-4e70-8857-ce00fc62fffb\Raspberry Pi 3298.ipt
- z:\worker\convert-fusion-r02-cosv3\tmp\job-1\86\output\files\932a8257-b544-4e70-8857-ce00fc62fffb\Raspberry Pi 3299.ipt
- z:\worker\convert-fusion-r02-cosv3\tmp\job-1\86\output\files\932a8257-b544-4e70-8857-ce00fc62fffb\Raspberry Pi 3300.ipt
- z:\worker\convert-fusion-r02-cosv3\tmp\job-1\86\output\files\932a8257-b544-4e70-8857-ce00fc62fffb\Raspberry Pi 3301.ipt
- z:\worker\convert-fusion-r02-cosv3\tmp\job-1\86\output\files\932a8257-b544-4e70-8857-ce00fc62fffb\Raspberry Pi 3302.ipt
- z:\worker\convert-fusion-r02-cosv3\tmp\job-1\86\output\files\932a8257-b544-4e70-8857-ce00fc62fffb\Raspberry Pi 3303.ipt
- z:\worker\convert-fusion-r02-cosv3\tmp\job-1\86\output\files\932a8257-b544-4e70-8857-ce00fc62fffb\Raspberry Pi 3304.ipt
- z:\worker\convert-fusion-r02-cosv3\tmp\job-1\86\output\files\932a8257-b544-4e70-8857-ce00fc62fffb\Raspberry Pi 3305.ipt
- z:\worker\convert-fusion-r02-cosv3\tmp\job-1\86\output\files\932a8257-b544-4e70-8857-ce00fc62fffb\Raspberry Pi 3306.ipt
- z:\worker\convert-fusion-r02-cosv3\tmp\job-1\86\output\files\932a8257-b544-4e70-8857-ce00fc62fffb\Raspberry Pi 3307.ipt
- z:\worker\convert-fusion-r02-cosv3\tmp\job-1\86\output\files\932a8257-b544-4e70-8857-ce00fc62fffb\Raspberry Pi 3308.ipt
- z:\worker\convert-fusion-r02-cosv3\tmp\job-1\86\output\files\932a8257-b544-4e70-8857-ce00fc62fffb\Raspberry Pi 3309.ipt
- z:\worker\convert-fusion-r02-cosv3\tmp\job-1\86\output\files\932a8257-b544-4e70-8857-ce00fc62fffb\Raspberry Pi 3310.ipt
- z:\worker\convert-fusion-r02-cosv3\tmp\job-1\86\output\files\932a8257-b544-4e70-8857-ce00fc62fffb\Raspberry Pi 3311.ipt
- z:\worker\convert-fusion-r02-cosv3\tmp\job-1\86\output\files\932a8257-b544-4e70-8857-ce00fc62fffb\Raspberry Pi 3312.ipt
- z:\worker\convert-fusion-r02-cosv3\tmp\job-1\86\output\files\932a8257-b544-4e70-8857-ce00fc62fffb\Raspberry Pi 3313.ipt
- z:\worker\convert-fusion-r02-cosv3\tmp\job-1\86\output\files\932a8257-b544-4e70-8857-ce00fc62fffb\Raspberry Pi 3314.ipt
- z:\worker\convert-fusion-r02-cosv3\tmp\job-1\86\output\files\932a8257-b544-4e70-8857-ce00fc62fffb\Raspberry Pi 3315.ipt
- z:\worker\convert-fusion-r02-cosv3\tmp\job-1\86\output\files\932a8257-b544-4e70-8857-ce00fc62fffb\Raspberry Pi 3316.ipt
- z:\worker\convert-fusion-r02-cosv3\tmp\job-1\86\output\files\932a8257-b544-4e70-8857-ce00fc62fffb\Raspberry Pi 3317.ipt
- z:\worker\convert-fusion-r02-cosv3\tmp\job-1\86\output\files\932a8257-b544-4e70-8857-ce00fc62fffb\Raspberry Pi 3318.ipt
- z:\worker\convert-fusion-r02-cosv3\tmp\job-1\86\output\files\932a8257-b544-4e70-8857-ce00fc62fffb\Raspberry Pi 3319.ipt
- z:\worker\convert-fusion-r02-cosv3\tmp\job-1\86\output\files\932a8257-b544-4e70-8857-ce00fc62fffb\Raspberry Pi 3320.ipt
- z:\worker\convert-fusion-r02-cosv3\tmp\job-1\86\output\files\932a8257-b544-4e70-8857-ce00fc62fffb\Raspberry Pi 3321.ipt
- z:\worker\convert-fusion-r02-cosv3\tmp\job-1\86\output\files\932a8257-b544-4e70-8857-ce00fc62fffb\Raspberry Pi 3322.ipt
- z:\worker\convert-fusion-r02-cosv3\tmp\job-1\86\output\files\932a8257-b544-4e70-8857-ce00fc62fffb\Raspberry Pi 3323.ipt
- z:\worker\convert-fusion-r02-cosv3\tmp\job-1\86\output\files\932a8257-b544-4e70-8857-ce00fc62fffb\Raspberry Pi 3324.ipt
- z:\worker\convert-fusion-r02-cosv3\tmp\job-1\86\output\files\932a8257-b544-4e70-8857-ce00fc62fffb\Raspberry Pi 3325.ipt
- z:\worker\convert-fusion-r02-cosv3\tmp\job-1\86\output\files\932a8257-b544-4e70-8857-ce00fc62fffb\Raspberry Pi 3326.ipt
- z:\worker\convert-fusion-r02-cosv3\tmp\job-1\86\output\files\932a8257-b544-4e70-8857-ce00fc62fffb\Raspberry Pi 3327.ipt
- z:\worker\convert-fusion-r02-cosv3\tmp\job-1\86\output\files\932a8257-b544-4e70-8857-ce00fc62fffb\Raspberry Pi 3328.ipt
- z:\worker\convert-fusion-r02-cosv3\tmp\job-1\86\output\files\932a8257-b544-4e70-8857-ce00fc62fffb\Raspberry Pi 3329.ipt
- z:\worker\convert-fusion-r02-cosv3\tmp\job-1\86\output\files\932a8257-b544-4e70-8857-ce00fc62fffb\Raspberry Pi 3330.ipt
- z:\worker\convert-fusion-r02-cosv3\tmp\job-1\86\output\files\932a8257-b544-4e70-8857-ce00fc62fffb\Raspberry Pi 3331.ipt
- z:\worker\convert-fusion-r02-cosv3\tmp\job-1\86\output\files\932a8257-b544-4e70-8857-ce00fc62fffb\Raspberry Pi 3332.ipt
- z:\worker\convert-fusion-r02-cosv3\tmp\job-1\86\output\files\932a8257-b544-4e70-8857-ce00fc62fffb\Raspberry Pi 3333.ipt
- z:\worker\convert-fusion-r02-cosv3\tmp\job-1\86\output\files\932a8257-b544-4e70-8857-ce00fc62fffb\Raspberry Pi 3334.ipt
- z:\worker\convert-fusion-r02-cosv3\tmp\job-1\86\output\files\932a8257-b544-4e70-8857-ce00fc62fffb\Raspberry Pi 3335.ipt
- z:\worker\convert-fusion-r02-cosv3\tmp\job-1\86\output\files\932a8257-b544-4e70-8857-ce00fc62fffb\Raspberry Pi 3336.ipt
- z:\worker\convert-fusion-r02-cosv3\tmp\job-1\86\output\files\932a8257-b544-4e70-8857-ce00fc62fffb\Raspberry Pi 3337.ipt
- z:\worker\convert-fusion-r02-cosv3\tmp\job-1\86\output\files\932a8257-b544-4e70-8857-ce00fc62fffb\Raspberry Pi 3338.ipt
- z:\worker\convert-fusion-r02-cosv3\tmp\job-1\86\output\files\932a8257-b544-4e70-8857-ce00fc62fffb\Raspberry Pi 3339.ipt
- z:\worker\convert-fusion-r02-cosv3\tmp\job-1\86\output\files\932a8257-b544-4e70-8857-ce00fc62fffb\Raspberry Pi 3340.ipt
- z:\worker\convert-fusion-r02-cosv3\tmp\job-1\86\output\files\932a8257-b544-4e70-8857-ce00fc62fffb\Raspberry Pi 3341.ipt
- z:\worker\convert-fusion-r02-cosv3\tmp\job-1\86\output\files\932a8257-b544-4e70-8857-ce00fc62fffb\Raspberry Pi 3342.ipt
- z:\worker\convert-fusion-r02-cosv3\tmp\job-1\86\output\files\932a8257-b544-4e70-8857-ce00fc62fffb\Raspberry Pi 3343.ipt
- z:\worker\convert-fusion-r02-cosv3\tmp\job-1\86\output\files\932a8257-b544-4e70-8857-ce00fc62fffb\Raspberry Pi 3344.ipt
- z:\worker\convert-fusion-r02-cosv3\tmp\job-1\86\output\files\932a8257-b544-4e70-8857-ce00fc62fffb\Raspberry Pi 3345.ipt
- z:\worker\convert-fusion-r02-cosv3\tmp\job-1\86\output\files\932a8257-b544-4e70-8857-ce00fc62fffb\Raspberry Pi 3346.ipt
- z:\worker\convert-fusion-r02-cosv3\tmp\job-1\86\output\files\932a8257-b544-4e70-8857-ce00fc62fffb\Raspberry Pi 3347.ipt
- z:\worker\convert-fusion-r02-cosv3\tmp\job-1\86\output\files\932a8257-b544-4e70-8857-ce00fc62fffb\Raspberry Pi 3348.ipt
- z:\worker\convert-fusion-r02-cosv3\tmp\job-1\86\output\files\932a8257-b544-4e70-8857-ce00fc62fffb\Raspberry Pi 3349.ipt
- z:\worker\convert-fusion-r02-cosv3\tmp\job-1\86\output\files\932a8257-b544-4e70-8857-ce00fc62fffb\Raspberry Pi 3350.ipt
- z:\worker\convert-fusion-r02-cosv3\tmp\job-1\86\output\files\932a8257-b544-4e70-8857-ce00fc62fffb\Raspberry Pi 3351.ipt
- z:\worker\convert-fusion-r02-cosv3\tmp\job-1\86\output\files\932a8257-b544-4e70-8857-ce00fc62fffb\Raspberry Pi 3352.ipt
- z:\worker\convert-fusion-r02-cosv3\tmp\job-1\86\output\files\932a8257-b544-4e70-8857-ce00fc62fffb\Raspberry Pi 3353.ipt
- z:\worker\convert-fusion-r02-cosv3\tmp\job-1\86\output\files\932a8257-b544-4e70-8857-ce00fc62fffb\Raspberry Pi 3354.ipt
- z:\worker\convert-fusion-r02-cosv3\tmp\job-1\86\output\files\932a8257-b544-4e70-8857-ce00fc62fffb\Raspberry Pi 3357.ipt
- z:\worker\convert-fusion-r02-cosv3\tmp\job-1\86\output\files\932a8257-b544-4e70-8857-ce00fc62fffb\Raspberry Pi 3355.ipt
- z:\worker\convert-fusion-r02-cosv3\tmp\job-1\86\output\files\932a8257-b544-4e70-8857-ce00fc62fffb\Raspberry Pi 3356.ipt
- z:\worker\convert-fusion-r02-cosv3\tmp\job-1\86\output\files\932a8257-b544-4e70-8857-ce00fc62fffb\Part2^Raspberry Pi 3.ipt
- z:\worker\convert-fusion-r02-cosv3\tmp\job-1\86\output\files\932a8257-b544-4e70-8857-ce00fc62fffb\Raspberry Pi 3360.ipt
- z:\worker\convert-fusion-r02-cosv3\tmp\job-1\86\output\files\932a8257-b544-4e70-8857-ce00fc62fffb\Part4^Raspberry Pi 3.ipt
- z:\worker\convert-fusion-r02-cosv3\tmp\job-1\86\output\files\932a8257-b544-4e70-8857-ce00fc62fffb\raspberry_pi_B+_(bar_180_2x20).ipt
- z:\worker\convert-fusion-r02-cosv3\tmp\job-1\86\output\files\932a8257-b544-4e70-8857-ce00fc62fffb\Solder2.ipt
- z:\worker\convert-fusion-r02-cosv3\tmp\job-1\86\output\files\932a8257-b544-4e70-8857-ce00fc62fffb\Solder2_Big.ipt
- z:\worker\convert-fusion-r02-cosv3\tmp\job-1\86\output\files\932a8257-b544-4e70-8857-ce00fc62fffb\Solder2_Small.ipt
- z:\worker\convert-fusion-r02-cosv3\tmp\job-1\86\output\files\932a8257-b544-4e70-8857-ce00fc62fffb\Raspberry Pi 3359.ipt
- z:\worker\convert-fusion-r02-cosv3\tmp\job-1\86\output\files\932a8257-b544-4e70-8857-ce00fc62fffb\mf-msmf050-2.ipt
- z:\worker\convert-fusion-r02-cosv3\tmp\job-1\86\output\files\932a8257-b544-4e70-8857-ce00fc62fffb\Raspberry Pi 3163_smaller.ipt
- z:\worker\convert-fusion-r02-cosv3\tmp\job-1\86\output\files\932a8257-b544-4e70-8857-ce00fc62fffb\Raspberry Pi 353_smaller.ipt
- z:\worker\convert-fusion-r02-cosv3\tmp\job-1\86\output\files\932a8257-b544-4e70-8857-ce00fc62fffb\Raspberry Pi 3164_small.ipt
- z:\worker\convert-fusion-r02-cosv3\tmp\job-1\86\output\files\932a8257-b544-4e70-8857-ce00fc62fffb\Raspberry Pi 3165_smaller.ipt
- z:\worker\convert-fusion-r02-cosv3\tmp\job-1\86\output\files\932a8257-b544-4e70-8857-ce00fc62fffb\Raspberry Pi 3141_smaller.ipt
- z:\worker\convert-fusion-r02-cosv3\tmp\job-1\86\output\files\932a8257-b544-4e70-8857-ce00fc62fffb\Part1^Raspberry Pi 3.ipt
- z:\worker\convert-fusion-r02-cosv3\tmp\job-1\86\output\files\932a8257-b544-4e70-8857-ce00fc62fffb\MOUNT.ipt
- z:\worker\convert-fusion-r02-cosv3\tmp\job-1\86\output\files\932a8257-b544-4e70-8857-ce00fc62fffb\94510A370_Brass Screw-to-Expand Inserts.ipt
- z:\worker\convert-fusion-r02-cosv3\tmp\job-1\86\output\files\932a8257-b544-4e70-8857-ce00fc62fffb\94209A347_Thread-Forming Screws for Soft Metal.ipt
## Components (642 placed, 369 different names)
1. Raspberry Pi 3157:1
2. Raspberry Pi 3236:1
3. Raspberry Pi 3237:1
4. Raspberry Pi 3238:1
5. Raspberry Pi 3239:1
6. Raspberry Pi 3240:1
7. Raspberry Pi 3241:1
8. Raspberry Pi 3242:1
9. Raspberry Pi 3243:1
10. Raspberry Pi 3244:1
11. Raspberry Pi 3245:1
12. Raspberry Pi 3246:1
13. Raspberry Pi 3247:1
14. Raspberry Pi 3248:1
15. Raspberry Pi 3249:1
16. Raspberry Pi 3250:1
17. Raspberry Pi 3251:1
18. Raspberry Pi 3252:1
19. Raspberry Pi 3253:1
20. Raspberry Pi 3254:1
21. Raspberry Pi 3255:1
22. Raspberry Pi 3256:1
23. Raspberry Pi 3257:1
24. Raspberry Pi 3258:1
25. Raspberry Pi 3259:1
26. Raspberry Pi 3260:1
27. Raspberry Pi 3261:1
28. Raspberry Pi 3262:1
29. Raspberry Pi 3263:1
30. Raspberry Pi 3264:1
31. Raspberry Pi 3265:1
32. Raspberry Pi 3266:1
33. Raspberry Pi 3267:1
34. Raspberry Pi 3268:1
35. Raspberry Pi 3269:1
36. Raspberry Pi 3270:1
37. Raspberry Pi 3271:1
38. Raspberry Pi 3272:1
39. Raspberry Pi 3273:1
40. Raspberry Pi 3274:1
41. Raspberry Pi 3275:1
42. RPi3_ModelB v1:1 [sub-assembly]
43. Raspberry Pi 312:1
44. Raspberry Pi 314:1
45. Raspberry Pi 3172:1
46. Raspberry Pi 3173:1
47. Raspberry Pi 3174:1
48. Raspberry Pi 3175:1
49. Raspberry Pi 3176:1
50. Raspberry Pi 3177:1
51. Raspberry Pi 3178:1
52. Raspberry Pi 3179:1
53. Raspberry Pi 3180:1
54. Raspberry Pi 3181:1
55. Raspberry Pi 3182:1
56. Raspberry Pi 3183:1
57. Raspberry Pi 3184:1
58. Raspberry Pi 3185:1
59. Raspberry Pi 3186:1
60. Raspberry Pi 3187:1
61. Raspberry Pi 3188:1
62. Raspberry Pi 3189:1
63. Raspberry Pi 3190:1
64. Raspberry Pi 3191:1
65. Raspberry Pi 3192:1
66. Raspberry Pi 3193:1
67. Raspberry Pi 3194:1
68. Raspberry Pi 3195:1
69. Raspberry Pi 3196:1
70. Raspberry Pi 3197:1
71. Raspberry Pi 3198:1
72. Raspberry Pi 3199:1
73. Raspberry Pi 3200:1
74. Raspberry Pi 3201:1
75. Raspberry Pi 3202:1
76. Raspberry Pi 3203:1
77. Raspberry Pi 3204:1
78. Raspberry Pi 3205:1
79. Raspberry Pi 3206:1
80. Raspberry Pi 3207:1
81. Raspberry Pi 3208:1
82. Raspberry Pi 3209:1
83. Raspberry Pi 3210:1
84. Raspberry Pi 3211:1
85. Raspberry Pi 3212:1
86. Raspberry Pi 3213:1
87. Raspberry Pi 3214:1
88. Raspberry Pi 3215:1
89. Raspberry Pi 3216:1
90. Raspberry Pi 3217:1
91. Raspberry Pi 3218:1
92. Raspberry Pi 3219:1
93. Raspberry Pi 3220:1
94. Raspberry Pi 3221:1
95. Raspberry Pi 3222:1
96. Raspberry Pi 3223:1
97. Raspberry Pi 3224:1
98. Raspberry Pi 3225:1
99. Raspberry Pi 3226:1
100. Raspberry Pi 3227:1
101. Raspberry Pi 3228:1
102. Raspberry Pi 3229:1
103. Raspberry Pi 3230:1
104. Raspberry Pi 3231:1
105. Raspberry Pi 3232:1
106. Raspberry Pi 3233:1
107. Raspberry Pi 3234:1
108. Raspberry Pi 3235:1
109. Raspberry Pi 31:1
110. Raspberry Pi 32:1
111. Raspberry Pi 33:1
112. Raspberry Pi 34:1
113. Raspberry Pi 35:1
114. Raspberry Pi 36:1
115. Raspberry Pi 37:1
116. Raspberry Pi 38:1
117. Raspberry Pi 39:1
118. Raspberry Pi 310:1
119. Raspberry Pi 311:1
120. Raspberry Pi 313:1
121. Raspberry Pi 315:1
122. Raspberry Pi 316:1
123. Raspberry Pi 317:1
124. Raspberry Pi 318:1
125. Raspberry Pi 319:1
126. Raspberry Pi 320:1
127. Raspberry Pi 322:1
128. Raspberry Pi 323:1
129. Raspberry Pi 324:1
130. Raspberry Pi 325:1
131. Raspberry Pi 326:1
132. Raspberry Pi 327:1
133. Raspberry Pi 328:1
134. Raspberry Pi 329:1
135. Raspberry Pi 330:1
136. Raspberry Pi 331:1
137. Raspberry Pi 332:1
138. Raspberry Pi 333:1
139. Raspberry Pi 334:1
140. Raspberry Pi 335:1
141. Raspberry Pi 336:1
142. Raspberry Pi 337:1
143. Raspberry Pi 338:1
144. Raspberry Pi 339:1
145. Raspberry Pi 340:1
146. Raspberry Pi 341:1
147. Raspberry Pi 342:1
148. Raspberry Pi 343:1
149. Raspberry Pi 344:1
150. Raspberry Pi 345:1
151. Raspberry Pi 346:1
152. Raspberry Pi 347:1
153. Raspberry Pi 348:1
154. Raspberry Pi 349:1
155. Raspberry Pi 350:1
156. Raspberry Pi 351:1
157. Raspberry Pi 352:1
158. Raspberry Pi 353:1
159. Raspberry Pi 354:1
160. Raspberry Pi 355:1
161. Raspberry Pi 356:1
162. Raspberry Pi 357:1
163. Raspberry Pi 358:1
164. Raspberry Pi 359:1
165. Raspberry Pi 360:1
166. Raspberry Pi 361:1
167. Raspberry Pi 362:1
168. Raspberry Pi 363:1
169. Raspberry Pi 364:1
170. Raspberry Pi 365:1
171. Raspberry Pi 366:1
172. Raspberry Pi 367:1
173. Raspberry Pi 368:1
174. Raspberry Pi 369:1
175. Raspberry Pi 370:1
176. Raspberry Pi 371:1
177. Raspberry Pi 372:1
178. Raspberry Pi 373:1
179. Raspberry Pi 374:1
180. Raspberry Pi 375:1
181. Raspberry Pi 376:1
182. Raspberry Pi 377:1
183. Raspberry Pi 378:1